# Autodesk Inventor assembly: Elbow
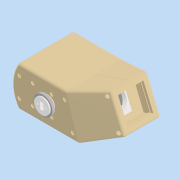
[picture p0: Inventor's stored thumbnail of the model, 180x180]
Saved by Autodesk Inventor 2021 (Build 250183000, 183)
## iProperties
Created: 2020-02-08
Part Number: Elbow
Document SubType Name: Assembly
Designer: JochenAlt
Author: JochenAlt
## Documents named in this file (5)
- C:\Users\Jochen Alt\Documents\Daten\Projects\MiniBot\CAD\Elbow.iam
- C:\Users\Jochen Alt\Documents\Daten\Projects\MiniBot\CAD\Elbow.ipt
- C:\Users\Jochen Alt\Documents\Daten\Projects\MiniBot\CAD\extern\Herkulex\Herkulex DRS-020x.ipt
- C:\Users\Jochen Alt\Documents\Daten\Projects\MiniBot\CAD\extern\Herkulex\Herkulex DRS-060x.ipt
- C:\Users\Jochen Alt\Documents\Daten\Projects\MiniBot\CAD\extern\bearings\20x27x4\W 61704-2ZS.iam
## Components (4 placed, 4 different names)
1. Elbow:1 — Winkel:3, Fluchtend:5, Passend:11, Passend:12, Passend:15, Winkel:4, Passend:17
2. Herkulex DRS-0201:1 — Winkel:4, Passend:17, Passend:18
3. Herkulex DRS-060x:1 — Winkel:3, Fluchtend:5, Passend:15, Passend:18
4. W 61704-2ZS:1 [sub-assembly] — Passend:11, Passend:12
## Relationships (8: Mate 5, Angle 2, Flush 1)
- Winkel:3 [Angle] (90 deg): Elbow:1 ↔ Herkulex DRS-060x:1
- Fluchtend:5 [Flush]: Elbow:1 ↔ Herkulex DRS-060x:1
- Passend:11 [Mate]: Elbow:1 ↔ W 61704-2ZS:1
- Passend:12 [Mate]: Elbow:1 ↔ W 61704-2ZS:1
- Passend:15 [Mate]: Elbow:1 ↔ Herkulex DRS-060x:1
- Winkel:4 [Angle] (180 deg): Elbow:1 ↔ Herkulex DRS-0201:1
- Passend:17 [Mate]: Elbow:1 ↔ Herkulex DRS-0201:1
- Passend:18 [Mate] (0.5 mm): Herkulex DRS-0201:1 ↔ Herkulex DRS-060x:1
